# Autodesk Inventor assembly: A1-19027-300-00 Spool SP-235-002-D-002-1
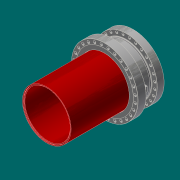
[picture p0: Inventor's stored thumbnail of the model, 180x180]
Saved by Autodesk Inventor 2017.3 (Build 213257000, 257)
## iProperties
Created: 2019-09-12
Part Number: A1-19027-300-00 Spool SP-235-002-D-002-1
Document SubType Name: Weldment
Designer: GVD
Weld Material: Steel, Mild, Welded
Mass: 1.25977e+06 g
Surface Area: 114700 cm^2
Volume: 165892 cm^3
Density: 7.59393 g/cm^3
Author: GVD
## Documents named in this file (6)
- N:\A1 - Projects\A1-19\A1-19027--Syncrude Aurora HT2 spools - SP-237\A1-19027-300-00 Spool SP-235-002-D-002-1.iam
- N:\A1 - Projects\A1-19\A1-19027--Syncrude Aurora HT2 spools - SP-237\A1-19027-300-01 32in pipe.ipt
- N:\A1 - Projects\A1-19\A1-19027--Syncrude Aurora HT2 spools - SP-237\A1-19027-300-02 32in CL150 RF flange.ipt
- N:\A1 - Projects\A1-19\A1-19027--Syncrude Aurora HT2 spools - SP-237\A1-19027-300-04 HCWI liner - nozzle.ipt
- N:\Penticton Foundry\Tag mount - 3in.ipt
- N:\A1 - Projects\A1-19\A1-19027--Syncrude Aurora HT2 spools - SP-237\A1-19027-300-03 Alco flange - 30in CL150.ipt
## Components (6 placed, 5 different names)
1. A1-19027-300-01 32in pipe:1 — Mate:2, Angle:1, Insert:1, Insert:2, Angle:3, Angle:4, Flush:1, Tangent:1
2. A1-19027-300-02 32in CL150 RF flange:1 — Insert:2, Angle:3
3. A1-19027-300-03 Alco flange - 30in CL150:1 — Mate:1, Insert:1, Insert:3, Flush:2
4. A1-19027-300-04 HCWI liner - nozzle:1 — Insert:3, Angle:4
5. A1-18023-150-08 Tag mount:1 — Flush:1, Flush:2, Tangent:1
6. A1-18023-150-08 Tag mount:2
## Component patterns: (2 elements, first: A1-18023-150-08 Tag mount:1)
## Relationships (12: Angle 4, Insert 3, Mate 2, Flush 2, Tangent 1)
- Mate:1: A1-19027-300-03 Alco flange - 30in CL150:1
- Mate:2: A1-19027-300-01 32in pipe:1
- Angle:1 (0 deg): A1-19027-300-01 32in pipe:1
- Insert:1 (2.3813 mm): A1-19027-300-01 32in pipe:1 ↔ A1-19027-300-03 Alco flange - 30in CL150:1
- [Angle] (0 deg): A1-19027-300-01 32in pipe:1 ↔ A1-19027-300-03 Alco flange - 30in CL150:1
- Insert:2 (2.3813 mm): A1-19027-300-01 32in pipe:1 ↔ A1-19027-300-02 32in CL150 RF flange:1
- Angle:3 (0 deg): A1-19027-300-01 32in pipe:1 ↔ A1-19027-300-02 32in CL150 RF flange:1
- Insert:3: A1-19027-300-03 Alco flange - 30in CL150:1 ↔ A1-19027-300-04 HCWI liner - nozzle:1
- Angle:4 (0 deg): A1-19027-300-01 32in pipe:1 ↔ A1-19027-300-04 HCWI liner - nozzle:1
- Flush:1: A1-19027-300-01 32in pipe:1 ↔ A1-18023-150-08 Tag mount:1
- Flush:2 (215.9 mm): A1-19027-300-03 Alco flange - 30in CL150:1 ↔ A1-18023-150-08 Tag mount:1
- Tangent:1: A1-19027-300-01 32in pipe:1 ↔ A1-18023-150-08 Tag mount:1
